# Autodesk Inventor assembly: GP3-100
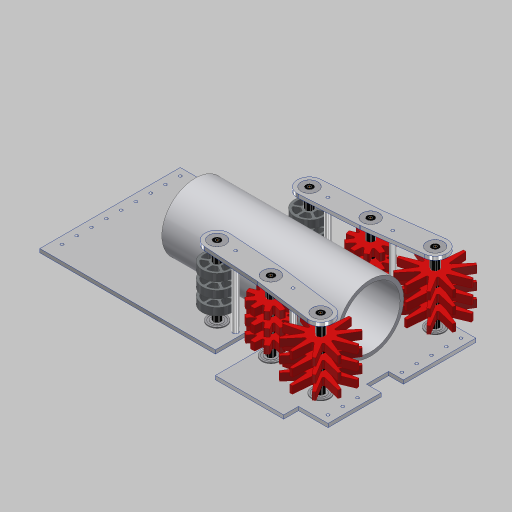
[picture p0: Inventor's stored thumbnail of the model, 512x512]
Saved by Autodesk Inventor 2023.5 (Build 275446000, 446)
## iProperties
Created: 2025-02-22
Part Number: GP3-100
Document SubType Name: Assembly
Designer: slick
Author: slick
## Documents named in this file (10)
- C:\Users\slick\OneDrive\Desktop\2025-ReefScape---CAD\ground intake\GP3\GP3-100.iam
- C:\Users\slick\OneDrive\Desktop\2025-ReefScape---CAD\ground intake\GP3\GP3-001.ipt
- C:\Users\slick\OneDrive\Desktop\2025-ReefScape---CAD\COMMON PARTS\BEARINGS\0_500_ID_x_1_125_OD_x_0_313_WD_Flanged_Bearing_217-2731.ipt
- C:\Users\slick\OneDrive\Desktop\2025-ReefScape---CAD\ground intake\GP3\GP3-002.ipt
- C:\Users\slick\OneDrive\Desktop\2025-ReefScape---CAD\COMMON PARTS\WHEELS\am-0619a .425 Hex Entrapption Star Cut to 4In.ipt
- C:\Users\slick\OneDrive\Desktop\2025-ReefScape---CAD\COMMON PARTS\WHEELS\am-0619a .425 Hex Entrapption Star Cut to 2 half In.ipt
- C:\Users\slick\OneDrive\Desktop\2025-ReefScape---CAD\COMMON PARTS\WHEELS\2_OD_Straight_Flex_Wheel_217-6354.ipt
- C:\Users\slick\OneDrive\Desktop\2025-ReefScape---CAD\ground intake\GP3\GP3-003.ipt
- C:\Users\slick\OneDrive\Desktop\2025-ReefScape---CAD\ground intake\GP3\GP3-004.ipt
- C:\Users\slick\OneDrive\Desktop\2025-ReefScape---CAD\Field Items\Game Pieces\GE-25500.ipt
## Components (44 placed, 9 different names)
1. GP3-001:1 — Insert:1, Insert:2, Insert:3, Mate:6, Insert:4, Insert:5, Insert:6, Insert:7, Insert:8, Insert:9, Insert:10, Tangent:1
2. 0_500_ID_x_1_125_OD_x_0_313_WD_Flanged_Bearing_217-2731:1 — Insert:2, Mate:2, Flush:2
3. 0_500_ID_x_1_125_OD_x_0_313_WD_Flanged_Bearing_217-2731:2 — Insert:1, Mate:3, Flush:1
4. 0_500_ID_x_1_125_OD_x_0_313_WD_Flanged_Bearing_217-2731:3 — Insert:3, Mate:1, Flush:3
5. GP3-002:1 — Mate:3, Flush:1, Mate:5
6. GP3-002:2 — Mate:1, Flush:3, Mate:4
7. GP3-002:3 — Mate:2, Flush:2, Mate:8
8. 0_500_ID_x_1_125_OD_x_0_313_WD_Flanged_Bearing_217-2731:4 — Insert:4
9. GP3-002:4 — Mate:9
10. 0_500_ID_x_1_125_OD_x_0_313_WD_Flanged_Bearing_217-2731:5 — Insert:5
11. GP3-002:5 — Mate:12
12. 0_500_ID_x_1_125_OD_x_0_313_WD_Flanged_Bearing_217-2731:6 — Insert:6
13. GP3-002:6 — Mate:13
14. GP3-003:1 — Insert:7, Insert:13
15. GP3-003:2 — Insert:8, Insert:14
16. GP3-003:3 — Insert:9, Insert:11
17. GP3-003:4 — Insert:10, Insert:12
18. GP3-004:1 — Insert:11, Insert:12, Insert:15, Insert:16, Insert:17
19. GP3-004:2 — Insert:13, Insert:14, Insert:18, Insert:19, Insert:20
20. 0_500_ID_x_1_125_OD_x_0_313_WD_Flanged_Bearing_217-2731:7 — Insert:18
21. 0_500_ID_x_1_125_OD_x_0_313_WD_Flanged_Bearing_217-2731:8 — Insert:15
22. 0_500_ID_x_1_125_OD_x_0_313_WD_Flanged_Bearing_217-2731:9 — Insert:20
23. 0_500_ID_x_1_125_OD_x_0_313_WD_Flanged_Bearing_217-2731:10 — Insert:17
24. 0_500_ID_x_1_125_OD_x_0_313_WD_Flanged_Bearing_217-2731:11 — Insert:16
25. 0_500_ID_x_1_125_OD_x_0_313_WD_Flanged_Bearing_217-2731:12 — Insert:19
26. GE-25500:1 — Tangent:1, Tangent:2
27. am-0619a .425 Hex Entrapption Star Cut to 4In:1 — Mate:4, Flush:4, Mate:6, Flush:7
28. am-0619a .425 Hex Entrapption Star Cut to 2 half In:2 — Mate:9, Flush:6, Flush:7, Flush:11
29. 2_OD_Straight_Flex_Wheel_217-6354:2 — Mate:12, Flush:10, Flush:11
30. 2_OD_Straight_Flex_Wheel_217-6354:1 — Mate:13, Flush:10
31. am-0619a .425 Hex Entrapption Star Cut to 2 half In:1 — Mate:8, Flush:6
32. am-0619a .425 Hex Entrapption Star Cut to 4In:2 — Mate:5, Flush:4
33. am-0619a .425 Hex Entrapption Star Cut to 4In:3
34. am-0619a .425 Hex Entrapption Star Cut to 2 half In:3
35. 2_OD_Straight_Flex_Wheel_217-6354:3
36. 2_OD_Straight_Flex_Wheel_217-6354:4 — Tangent:2
37. am-0619a .425 Hex Entrapption Star Cut to 2 half In:4
38. am-0619a .425 Hex Entrapption Star Cut to 4In:4
39. am-0619a .425 Hex Entrapption Star Cut to 4In:5
40. am-0619a .425 Hex Entrapption Star Cut to 2 half In:5
41. 2_OD_Straight_Flex_Wheel_217-6354:5
42. 2_OD_Straight_Flex_Wheel_217-6354:6
43. am-0619a .425 Hex Entrapption Star Cut to 2 half In:6
44. am-0619a .425 Hex Entrapption Star Cut to 4In:6
## Component patterns: (3 elements, first: am-0619a .425 Hex Entrapption Star Cut to 4In:1 + am-0619a .425 Hex Entrapption Star Cut to 2 half In:2 + 2_OD_Straight_Flex_Wheel_217-6354:2 + 2_OD_Straight_Flex_Wheel_217-6354:1 + am-0619a .425 Hex Entrapption Star Cut to 2 half In:1 + am-0619a .425 Hex Entrapption Star Cut to 4In:2)
## Relationships (46: Insert 20, Mate 13, Flush 11, Tangent 2)
- Insert:1: GP3-001:1 ↔ 0_500_ID_x_1_125_OD_x_0_313_WD_Flanged_Bearing_217-2731:2
- Insert:2: GP3-001:1 ↔ 0_500_ID_x_1_125_OD_x_0_313_WD_Flanged_Bearing_217-2731:1
- Insert:3: GP3-001:1 ↔ 0_500_ID_x_1_125_OD_x_0_313_WD_Flanged_Bearing_217-2731:3
- Mate:1: 0_500_ID_x_1_125_OD_x_0_313_WD_Flanged_Bearing_217-2731:3 ↔ GP3-002:2
- Mate:2: 0_500_ID_x_1_125_OD_x_0_313_WD_Flanged_Bearing_217-2731:1 ↔ GP3-002:3
- Mate:3: 0_500_ID_x_1_125_OD_x_0_313_WD_Flanged_Bearing_217-2731:2 ↔ GP3-002:1
- Flush:1: 0_500_ID_x_1_125_OD_x_0_313_WD_Flanged_Bearing_217-2731:2 ↔ GP3-002:1
- Flush:2: 0_500_ID_x_1_125_OD_x_0_313_WD_Flanged_Bearing_217-2731:1 ↔ GP3-002:3
- Flush:3: 0_500_ID_x_1_125_OD_x_0_313_WD_Flanged_Bearing_217-2731:3 ↔ GP3-002:2
- Mate:4: GP3-002:2 ↔ am-0619a .425 Hex Entrapption Star Cut to 4In:1
- Mate:5: GP3-002:1 ↔ am-0619a .425 Hex Entrapption Star Cut to 4In:2
- Flush:4: am-0619a .425 Hex Entrapption Star Cut to 4In:1 ↔ am-0619a .425 Hex Entrapption Star Cut to 4In:2
- Mate:6 (25.4 mm): GP3-001:1 ↔ am-0619a .425 Hex Entrapption Star Cut to 4In:1
- [Mate]: 0_500_ID_x_1_125_OD_x_0_313_WD_Flanged_Bearing_217-2731:4 ↔ GP3-002:4
- [Flush]: 0_500_ID_x_1_125_OD_x_0_313_WD_Flanged_Bearing_217-2731:4 ↔ GP3-002:4
- Insert:4: GP3-001:1 ↔ 0_500_ID_x_1_125_OD_x_0_313_WD_Flanged_Bearing_217-2731:4
- Mate:8: GP3-002:3 ↔ am-0619a .425 Hex Entrapption Star Cut to 2 half In:1
- Mate:9: GP3-002:4 ↔ am-0619a .425 Hex Entrapption Star Cut to 2 half In:2
- Flush:6: am-0619a .425 Hex Entrapption Star Cut to 2 half In:2 ↔ am-0619a .425 Hex Entrapption Star Cut to 2 half In:1
- Flush:7: am-0619a .425 Hex Entrapption Star Cut to 4In:1 ↔ am-0619a .425 Hex Entrapption Star Cut to 2 half In:2
- [Mate]: 0_500_ID_x_1_125_OD_x_0_313_WD_Flanged_Bearing_217-2731:5 ↔ GP3-002:5
- [Flush]: 0_500_ID_x_1_125_OD_x_0_313_WD_Flanged_Bearing_217-2731:5 ↔ GP3-002:5
- [Mate]: 0_500_ID_x_1_125_OD_x_0_313_WD_Flanged_Bearing_217-2731:6 ↔ GP3-002:6
- [Flush]: 0_500_ID_x_1_125_OD_x_0_313_WD_Flanged_Bearing_217-2731:6 ↔ GP3-002:6
- Insert:5: GP3-001:1 ↔ 0_500_ID_x_1_125_OD_x_0_313_WD_Flanged_Bearing_217-2731:5
- Insert:6: GP3-001:1 ↔ 0_500_ID_x_1_125_OD_x_0_313_WD_Flanged_Bearing_217-2731:6
- Mate:12: GP3-002:5 ↔ 2_OD_Straight_Flex_Wheel_217-6354:2
- Mate:13: GP3-002:6 ↔ 2_OD_Straight_Flex_Wheel_217-6354:1
- Flush:10: 2_OD_Straight_Flex_Wheel_217-6354:2 ↔ 2_OD_Straight_Flex_Wheel_217-6354:1
- Flush:11: am-0619a .425 Hex Entrapption Star Cut to 2 half In:2 ↔ 2_OD_Straight_Flex_Wheel_217-6354:2
- Insert:7: GP3-001:1 ↔ GP3-003:1
- Insert:8: GP3-001:1 ↔ GP3-003:2
- Insert:9: GP3-001:1 ↔ GP3-003:3
- Insert:10: GP3-001:1 ↔ GP3-003:4
- Insert:11: GP3-003:3 ↔ GP3-004:1
- Insert:12: GP3-003:4 ↔ GP3-004:1
- Insert:13: GP3-003:1 ↔ GP3-004:2
- Insert:14: GP3-003:2 ↔ GP3-004:2
- Insert:15: GP3-004:1 ↔ 0_500_ID_x_1_125_OD_x_0_313_WD_Flanged_Bearing_217-2731:8
- Insert:16: GP3-004:1 ↔ 0_500_ID_x_1_125_OD_x_0_313_WD_Flanged_Bearing_217-2731:11
- Insert:17: GP3-004:1 ↔ 0_500_ID_x_1_125_OD_x_0_313_WD_Flanged_Bearing_217-2731:10
- Insert:18: GP3-004:2 ↔ 0_500_ID_x_1_125_OD_x_0_313_WD_Flanged_Bearing_217-2731:7
- Insert:19: GP3-004:2 ↔ 0_500_ID_x_1_125_OD_x_0_313_WD_Flanged_Bearing_217-2731:12
- Insert:20: GP3-004:2 ↔ 0_500_ID_x_1_125_OD_x_0_313_WD_Flanged_Bearing_217-2731:9
- Tangent:1: GP3-001:1 ↔ GE-25500:1
- Tangent:2 (-3.175 mm): GE-25500:1 ↔ 2_OD_Straight_Flex_Wheel_217-6354:4
## Named parameters: d26_d10 = 0 mm, d27_d7 = 0 mm, d33_d26_d10 = 0 mm, d34_d27_d7 = 0 mm, d35_d33_d26_d10 = 0 mm, d36_d34_d27_d7 = 0 mm
